# Autodesk Inventor assembly: Сборка
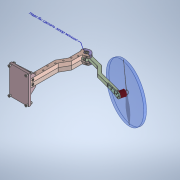
[picture p0: Inventor's stored thumbnail of the model, 180x180]
Saved by Autodesk Inventor 2021.2 (Build 252289000, 289)
## iProperties
Created: 2024-10-29
Part Number: Сборка
Document SubType Name: Assembly
Designer: barko
Author: barko
## Documents named in this file (24)
- C:\Users\DELL\Desktop\Personal\PID_controller\PID_controller\Mechanics\3D_model\Сборка.iam
- C:\Users\DELL\Desktop\Personal\PID_controller\PID_controller\Mechanics\3D_model\Ножка 1.ipt
- C:\Users\DELL\Desktop\Personal\PID_controller\PID_controller\Mechanics\3D_model\Ножка 2.ipt
- C:\Users\DELL\Desktop\Personal\PID_controller\PID_controller\Mechanics\3D_model\Скобка 1.ipt
- C:\Users\DELL\Desktop\Personal\PID_controller\PID_controller\Mechanics\3D_model\Скобка 2.ipt
- C:\Users\DELL\Desktop\Personal\PID_controller\PID_controller\Mechanics\3D_model\Фланец.ipt
- C:\Users\DELL\Desktop\Personal\PID_controller\PID_controller\Mechanics\3D_model\Луч.ipt
- C:\Users\DELL\Desktop\Personal\PID_controller\PID_controller\Mechanics\3D_model\Ложечка.ipt
- C:\Users\DELL\Desktop\Personal\PID_controller\PID_controller\Mechanics\3D_model\Моторчик.ipt
- C:\Users\DELL\Desktop\Personal\PID_controller\PID_controller\Mechanics\3D_model\Пропеллер.ipt
- C:\Users\DELL\Documents\Inventor\Content Center Files\R2021\ru-RU\GOST 11738-84\Винт M3-6gx30 ГОСТ 11738-84.ipt
- C:\Users\DELL\Documents\Inventor\Content Center Files\R2021\ru-RU\GOST 5916-70\Гайка M3-6H ГОСТ 5916-70.ipt
- C:\Users\DELL\Documents\Inventor\Content Center Files\R2021\ru-RU\Nut GOST 15524-70\Гайка M4-6H ГОСТ 15524-70.ipt
- C:\Users\DELL\Documents\Inventor\Content Center Files\R2021\ru-RU\GOST 11738-84\Винт M4-6gx25 ГОСТ 11738-84.ipt
- C:\Users\DELL\Documents\Inventor\Content Center Files\R2021\ru-RU\GOST 11738-84\Винт M4-6gx20 ГОСТ 11738-84.ipt
- C:\Users\DELL\Desktop\Personal\PID_controller\PID_controller\Mechanics\3D_model\Подшипник.ipt
- C:\Users\DELL\Documents\Inventor\Content Center Files\R2021\ru-RU\GOST 5915-70\Гайка M6-6H ГОСТ 5915-70(1).ipt
- C:\Users\DELL\Documents\Inventor\Content Center Files\R2021\ru-RU\GOST 11738-84\Винт M6-6gx50 ГОСТ 11738-84.ipt
- C:\Users\DELL\Documents\Inventor\Content Center Files\R2021\ru-RU\GOST 11738-84\Винт M6-6gx25 ГОСТ 11738-84.ipt
- C:\Users\DELL\Documents\Inventor\Content Center Files\R2021\ru-RU\GOST 11371-78  A\Шайба 6 ГОСТ 11371-78.ipt
- C:\Users\DELL\Documents\Inventor\Content Center Files\R2021\ru-RU\Washer 1 GOST 6402-78\Шайба 6Л ГОСТ 6402-78.ipt
- C:\Users\DELL\Documents\Inventor\Content Center Files\R2021\ru-RU\GOST 17475-80 (2)\Винт 2.M6-6gx30 ГОСТ 17475-80.ipt
- C:\Users\DELL\Documents\Inventor\Content Center Files\R2021\ru-RU\ISO 10642(1)\ISO 10642 - M3x8.ipt
- C:\Users\DELL\Documents\Inventor\Content Center Files\R2021\ru-RU\ISO 10642(1)\ISO 10642 - M3x12.ipt
## Components (68 placed, 23 different names)
1. Ножка 1:1 — Совмещение:1, Угол:1, Совмещение:2, Совмещение:3, Совмещение:4, Совмещение:5, Совмещение:6, Совмещение:7, Совмещение:8, Совмещение:9, Совмещение:10, Совмещение:11, Совмещение:12, Совмещение:13, Совмещение:14, Совмещение:15, Совмещение:16, Совмещение:18, Совмещение:20, Совмещение:22, Совмещение:24, Совмещение:26, Совмещение:28, Вставка:4, Совмещение:46, Совмещение:58, Совмещение:62, Совмещение:64
2. Ножка 2:1 — Совмещение:17, Совмещение:19, Совмещение:21, Совмещение:23, Совмещение:25, Совмещение:27, Совмещение:29, Вставка:5, Совмещение:59, Совмещение:60, Совмещение:63, Совмещение:65
3. Скобка 1:1 — Совмещение:42, Совмещение:43, Совмещение:44, Совмещение:53, Совмещение:54, Совмещение:55
4. Скобка 2:1 — Совмещение:47, Совмещение:48, Совмещение:49, Совмещение:50, Совмещение:51, Совмещение:52
5. Фланец:1 — Совмещение:66, Совмещение:67, Совмещение:68, Совмещение:69, Совмещение:70, Совмещение:71, Совмещение:72, Совмещение:73, Совмещение:74, Совмещение:75, Совмещение:76, Совмещение:77, Вставка:6, Вставка:7, Вставка:8, Вставка:9, Заподлицо:2, Заподлицо:3, Заподлицо:4, Заподлицо:5
6. Луч:1 — Заподлицо:1, Совмещение:1, Угол:1, Совмещение:37, Совмещение:38, Совмещение:40, Совмещение:41, Совмещение:95, Совмещение:96, Угол:2
7. Ложечка:1 — Вставка:1, Совмещение:86, Совмещение:87, Совмещение:88, Совмещение:89, Совмещение:90, Совмещение:91, Совмещение:92, Совмещение:93, Совмещение:94, Совмещение:96, Угол:2
8. Моторчик:1 — Вставка:1, Вставка:2, Совмещение:95
9. Пропеллер:1 — Вставка:2
10. Подшипник:1 — Вставка:4
11. Подшипник:2 — Вставка:5
12. Винт ГОСТ 11738-84 M 3x30:1 — Совмещение:2, Совмещение:3
13. Гайка ГОСТ 5916-70 M3:1 — Совмещение:16, Совмещение:17
14. Винт ГОСТ 11738-84 M 3x30:2 — Совмещение:4, Совмещение:5
15. Винт ГОСТ 11738-84 M 3x30:3 — Совмещение:6, Совмещение:7
16. Винт ГОСТ 11738-84 M 3x30:4 — Совмещение:8, Совмещение:9
17. Винт ГОСТ 11738-84 M 3x30:5 — Совмещение:10, Совмещение:11
18. Винт ГОСТ 11738-84 M 3x30:6 — Совмещение:12, Совмещение:13
19. Винт ГОСТ 11738-84 M 3x30:7 — Совмещение:14, Совмещение:15
20. Гайка ГОСТ 5916-70 M3:2 — Совмещение:18, Совмещение:19
21. Гайка ГОСТ 5916-70 M3:3 — Совмещение:20, Совмещение:21
22. Гайка ГОСТ 5916-70 M3:4 — Совмещение:22, Совмещение:23
23. Гайка ГОСТ 5916-70 M3:5 — Совмещение:24, Совмещение:25
24. Гайка ГОСТ 5916-70 M3:6 — Совмещение:26, Совмещение:27
25. Гайка ГОСТ 5916-70 M3:7 — Совмещение:28, Совмещение:29
26. Винт ГОСТ 11738-84 M 4x20:1 — Совмещение:45, Совмещение:46
27. Гайка ГОСТ 15524-70 M4:1 — Совмещение:42, Совмещение:43, Совмещение:44, Совмещение:45
28. Винт ГОСТ 11738-84 M 4x25:1 — Совмещение:37, Совмещение:39
29. Гайка ГОСТ 15524-70 M4:2 — Совмещение:38, Совмещение:39, Совмещение:40, Совмещение:41
30. Винт ГОСТ 11738-84 M 4x20:2 — Совмещение:56, Совмещение:58
31. Винт ГОСТ 11738-84 M 4x20:3 — Совмещение:60, Совмещение:61
32. Винт ГОСТ 11738-84 M 4x20:4 — Совмещение:57, Совмещение:59
33. Гайка ГОСТ 15524-70 M4:3 — Совмещение:47, Совмещение:48, Совмещение:49, Совмещение:61
34. Гайка ГОСТ 15524-70 M4:4 — Совмещение:53, Совмещение:54, Совмещение:55, Совмещение:56
35. Гайка ГОСТ 15524-70 M4:5 — Совмещение:50, Совмещение:51, Совмещение:52, Совмещение:57
36. Гайка ГОСТ 5915-70 M6:1 — Совмещение:69, Совмещение:72, Совмещение:73, Совмещение:80
37. Гайка ГОСТ 5915-70 M6:2 — Совмещение:71, Совмещение:74, Совмещение:75, Совмещение:81
38. Гайка ГОСТ 5915-70 M6:3 — Совмещение:70, Совмещение:76, Совмещение:77, Совмещение:79
39. Гайка ГОСТ 5915-70 M6:4 — Совмещение:66, Совмещение:67, Совмещение:68, Совмещение:78
40. Винт ГОСТ 11738-84 M 6x50:1 — Совмещение:64, Совмещение:79
41. Винт ГОСТ 11738-84 M 6x25:2 — Совмещение:63, Совмещение:80
42. Винт ГОСТ 11738-84 M 6x25:1 — Совмещение:62, Совмещение:78
43. Винт ГОСТ 11738-84 M 6x50:2 — Совмещение:65, Совмещение:81
44. Шайба  ГОСТ 11371-78 6,4:1 — Вставка:6, Вставка:10
45. Шайба  ГОСТ 11371-78 6,4:2 — Вставка:7, Вставка:11
46. Шайба  ГОСТ 11371-78 6,4:3 — Вставка:8, Вставка:13
47. Шайба  ГОСТ 11371-78 6,4:4 — Вставка:9, Вставка:12
48. Шайба 1 ГОСТ 6402-78 6Л:1 — Вставка:10, Вставка:16
49. Шайба 1 ГОСТ 6402-78 6Л:2 — Вставка:11, Вставка:15
50. Шайба 1 ГОСТ 6402-78 6Л:3 — Вставка:12, Вставка:17
51. Шайба 1 ГОСТ 6402-78 6Л:4 — Вставка:13, Вставка:14
52. Гайка ГОСТ 5915-70 M6:5 — Вставка:14, Совмещение:85
53. Гайка ГОСТ 5915-70 M6:6 — Вставка:15, Совмещение:84
54. Гайка ГОСТ 5915-70 M6:7 — Вставка:16, Совмещение:82
55. Гайка ГОСТ 5915-70 M6:8 — Вставка:17, Совмещение:83
56. Винт 2 ГОСТ 17475-80 M6 x 30:1 — Совмещение:82, Заподлицо:3
57. Винт 2 ГОСТ 17475-80 M6 x 30:2 — Совмещение:83, Заподлицо:2
58. Винт 2 ГОСТ 17475-80 M6 x 30:3 — Совмещение:85, Заподлицо:5
59. Винт 2 ГОСТ 17475-80 M6 x 30:4 — Совмещение:84, Заподлицо:4
60. ISO 10642 M3x12:1 — Совмещение:86
61. ISO 10642 M3x12:2 — Совмещение:87
62. ISO 10642 M3x12:3 — Совмещение:88
63. ISO 10642 M3x12:4 — Совмещение:89
64. ISO 10642 M3x12:5 — Совмещение:90
65. ISO 10642 M3x8:1 — Совмещение:91
66. ISO 10642 M3x8:2 — Совмещение:92
67. ISO 10642 M3x8:3 — Совмещение:93
68. ISO 10642 M3x8:4 — Совмещение:94
## Relationships (112: Mate 89, Insert 16, Flush 5, Angle 2)
- Вставка:1 [Insert]: Ложечка:1 ↔ Моторчик:1
- Вставка:2 [Insert] (2 mm): Моторчик:1 ↔ Пропеллер:1
- Заподлицо:1 [Flush]: Луч:1
- Совмещение:1 [Mate]: Ножка 1:1 ↔ Луч:1
- Угол:1 [Angle] (0 deg): Ножка 1:1 ↔ Луч:1
- Совмещение:2 [Mate]: Ножка 1:1 ↔ Винт ГОСТ 11738-84 M 3x30:1
- Совмещение:3 [Mate]: Ножка 1:1 ↔ Винт ГОСТ 11738-84 M 3x30:1
- Совмещение:4 [Mate]: Ножка 1:1 ↔ Винт ГОСТ 11738-84 M 3x30:2
- Совмещение:5 [Mate]: Ножка 1:1 ↔ Винт ГОСТ 11738-84 M 3x30:2
- Совмещение:6 [Mate]: Ножка 1:1 ↔ Винт ГОСТ 11738-84 M 3x30:3
- Совмещение:7 [Mate]: Ножка 1:1 ↔ Винт ГОСТ 11738-84 M 3x30:3
- Совмещение:8 [Mate]: Ножка 1:1 ↔ Винт ГОСТ 11738-84 M 3x30:4
- Совмещение:9 [Mate]: Ножка 1:1 ↔ Винт ГОСТ 11738-84 M 3x30:4
- Совмещение:10 [Mate]: Ножка 1:1 ↔ Винт ГОСТ 11738-84 M 3x30:5
- Совмещение:11 [Mate]: Ножка 1:1 ↔ Винт ГОСТ 11738-84 M 3x30:5
- Совмещение:12 [Mate]: Ножка 1:1 ↔ Винт ГОСТ 11738-84 M 3x30:6
- Совмещение:13 [Mate]: Ножка 1:1 ↔ Винт ГОСТ 11738-84 M 3x30:6
- Совмещение:14 [Mate]: Ножка 1:1 ↔ Винт ГОСТ 11738-84 M 3x30:7
- Совмещение:15 [Mate]: Ножка 1:1 ↔ Винт ГОСТ 11738-84 M 3x30:7
- Совмещение:16 [Mate]: Ножка 1:1 ↔ Гайка ГОСТ 5916-70 M3:1
- Совмещение:17 [Mate]: Ножка 2:1 ↔ Гайка ГОСТ 5916-70 M3:1
- Совмещение:18 [Mate]: Ножка 1:1 ↔ Гайка ГОСТ 5916-70 M3:2
- Совмещение:19 [Mate]: Ножка 2:1 ↔ Гайка ГОСТ 5916-70 M3:2
- Совмещение:20 [Mate]: Ножка 1:1 ↔ Гайка ГОСТ 5916-70 M3:3
- Совмещение:21 [Mate]: Ножка 2:1 ↔ Гайка ГОСТ 5916-70 M3:3
- Совмещение:22 [Mate]: Ножка 1:1 ↔ Гайка ГОСТ 5916-70 M3:4
- Совмещение:23 [Mate]: Ножка 2:1 ↔ Гайка ГОСТ 5916-70 M3:4
- Совмещение:24 [Mate]: Ножка 1:1 ↔ Гайка ГОСТ 5916-70 M3:5
- Совмещение:25 [Mate]: Ножка 2:1 ↔ Гайка ГОСТ 5916-70 M3:5
- Совмещение:26 [Mate]: Ножка 1:1 ↔ Гайка ГОСТ 5916-70 M3:6
- Совмещение:27 [Mate]: Ножка 2:1 ↔ Гайка ГОСТ 5916-70 M3:6
- Совмещение:28 [Mate]: Ножка 1:1 ↔ Гайка ГОСТ 5916-70 M3:7
- Совмещение:29 [Mate]: Ножка 2:1 ↔ Гайка ГОСТ 5916-70 M3:7
- Совмещение:37 [Mate]: Луч:1 ↔ Винт ГОСТ 11738-84 M 4x25:1
- Совмещение:38 [Mate]: Луч:1 ↔ Гайка ГОСТ 15524-70 M4:2
- Совмещение:39 [Mate]: Винт ГОСТ 11738-84 M 4x25:1 ↔ Гайка ГОСТ 15524-70 M4:2
- Совмещение:40 [Mate]: Луч:1 ↔ Гайка ГОСТ 15524-70 M4:2
- Совмещение:41 [Mate]: Луч:1 ↔ Гайка ГОСТ 15524-70 M4:2
- Вставка:4 [Insert]: Ножка 1:1 ↔ Подшипник:1
- Вставка:5 [Insert]: Ножка 2:1 ↔ Подшипник:2
- Совмещение:42 [Mate]: Скобка 1:1 ↔ Гайка ГОСТ 15524-70 M4:1
- Совмещение:43 [Mate]: Скобка 1:1 ↔ Гайка ГОСТ 15524-70 M4:1
- Совмещение:44 [Mate]: Скобка 1:1 ↔ Гайка ГОСТ 15524-70 M4:1
- Совмещение:45 [Mate]: Винт ГОСТ 11738-84 M 4x20:1 ↔ Гайка ГОСТ 15524-70 M4:1
- Совмещение:46 [Mate]: Ножка 1:1 ↔ Винт ГОСТ 11738-84 M 4x20:1
- Совмещение:47 [Mate]: Скобка 2:1 ↔ Гайка ГОСТ 15524-70 M4:3
- Совмещение:48 [Mate]: Скобка 2:1 ↔ Гайка ГОСТ 15524-70 M4:3
- Совмещение:49 [Mate]: Скобка 2:1 ↔ Гайка ГОСТ 15524-70 M4:3
- Совмещение:50 [Mate]: Скобка 2:1 ↔ Гайка ГОСТ 15524-70 M4:5
- Совмещение:51 [Mate]: Скобка 2:1 ↔ Гайка ГОСТ 15524-70 M4:5
- Совмещение:52 [Mate]: Скобка 2:1 ↔ Гайка ГОСТ 15524-70 M4:5
- Совмещение:53 [Mate]: Скобка 1:1 ↔ Гайка ГОСТ 15524-70 M4:4
- Совмещение:54 [Mate]: Скобка 1:1 ↔ Гайка ГОСТ 15524-70 M4:4
- Совмещение:55 [Mate]: Скобка 1:1 ↔ Гайка ГОСТ 15524-70 M4:4
- Совмещение:56 [Mate]: Винт ГОСТ 11738-84 M 4x20:2 ↔ Гайка ГОСТ 15524-70 M4:4
- Совмещение:57 [Mate]: Винт ГОСТ 11738-84 M 4x20:4 ↔ Гайка ГОСТ 15524-70 M4:5
- Совмещение:58 [Mate]: Ножка 1:1 ↔ Винт ГОСТ 11738-84 M 4x20:2
- Совмещение:59 [Mate]: Ножка 2:1 ↔ Винт ГОСТ 11738-84 M 4x20:4
- Совмещение:60 [Mate]: Ножка 2:1 ↔ Винт ГОСТ 11738-84 M 4x20:3
- Совмещение:61 [Mate]: Винт ГОСТ 11738-84 M 4x20:3 ↔ Гайка ГОСТ 15524-70 M4:3
- Совмещение:62 [Mate]: Ножка 1:1 ↔ Винт ГОСТ 11738-84 M 6x25:1
- Совмещение:63 [Mate]: Ножка 2:1 ↔ Винт ГОСТ 11738-84 M 6x25:2
- Совмещение:64 [Mate]: Ножка 1:1 ↔ Винт ГОСТ 11738-84 M 6x50:1
- Совмещение:65 [Mate]: Ножка 2:1 ↔ Винт ГОСТ 11738-84 M 6x50:2
- Совмещение:66 [Mate]: Фланец:1 ↔ Гайка ГОСТ 5915-70 M6:4
- Совмещение:67 [Mate]: Фланец:1 ↔ Гайка ГОСТ 5915-70 M6:4
- Совмещение:68 [Mate]: Фланец:1 ↔ Гайка ГОСТ 5915-70 M6:4
- Совмещение:69 [Mate]: Фланец:1 ↔ Гайка ГОСТ 5915-70 M6:1
- Совмещение:70 [Mate]: Фланец:1 ↔ Гайка ГОСТ 5915-70 M6:3
- Совмещение:71 [Mate]: Фланец:1 ↔ Гайка ГОСТ 5915-70 M6:2
- Совмещение:72 [Mate]: Фланец:1 ↔ Гайка ГОСТ 5915-70 M6:1
- Совмещение:73 [Mate]: Фланец:1 ↔ Гайка ГОСТ 5915-70 M6:1
- Совмещение:74 [Mate]: Фланец:1 ↔ Гайка ГОСТ 5915-70 M6:2
- Совмещение:75 [Mate]: Фланец:1 ↔ Гайка ГОСТ 5915-70 M6:2
- Совмещение:76 [Mate]: Фланец:1 ↔ Гайка ГОСТ 5915-70 M6:3
- Совмещение:77 [Mate]: Фланец:1 ↔ Гайка ГОСТ 5915-70 M6:3
- Совмещение:78 [Mate]: Гайка ГОСТ 5915-70 M6:4 ↔ Винт ГОСТ 11738-84 M 6x25:1
- Совмещение:79 [Mate]: Гайка ГОСТ 5915-70 M6:3 ↔ Винт ГОСТ 11738-84 M 6x50:1
- Совмещение:80 [Mate]: Гайка ГОСТ 5915-70 M6:1 ↔ Винт ГОСТ 11738-84 M 6x25:2
- Совмещение:81 [Mate]: Гайка ГОСТ 5915-70 M6:2 ↔ Винт ГОСТ 11738-84 M 6x50:2
- Вставка:6 [Insert]: Фланец:1 ↔ Шайба  ГОСТ 11371-78 6,4:1
- Вставка:7 [Insert]: Фланец:1 ↔ Шайба  ГОСТ 11371-78 6,4:2
- Вставка:8 [Insert]: Фланец:1 ↔ Шайба  ГОСТ 11371-78 6,4:3
- Вставка:9 [Insert]: Фланец:1 ↔ Шайба  ГОСТ 11371-78 6,4:4
- Вставка:10 [Insert]: Шайба  ГОСТ 11371-78 6,4:1 ↔ Шайба 1 ГОСТ 6402-78 6Л:1
- Вставка:11 [Insert]: Шайба  ГОСТ 11371-78 6,4:2 ↔ Шайба 1 ГОСТ 6402-78 6Л:2
- Вставка:12 [Insert]: Шайба  ГОСТ 11371-78 6,4:4 ↔ Шайба 1 ГОСТ 6402-78 6Л:3
- Вставка:13 [Insert]: Шайба  ГОСТ 11371-78 6,4:3 ↔ Шайба 1 ГОСТ 6402-78 6Л:4
- Вставка:14 [Insert]: Шайба 1 ГОСТ 6402-78 6Л:4 ↔ Гайка ГОСТ 5915-70 M6:5
- Вставка:15 [Insert]: Шайба 1 ГОСТ 6402-78 6Л:2 ↔ Гайка ГОСТ 5915-70 M6:6
- Вставка:16 [Insert]: Шайба 1 ГОСТ 6402-78 6Л:1 ↔ Гайка ГОСТ 5915-70 M6:7
- Вставка:17 [Insert]: Шайба 1 ГОСТ 6402-78 6Л:3 ↔ Гайка ГОСТ 5915-70 M6:8
- Совмещение:82 [Mate]: Гайка ГОСТ 5915-70 M6:7 ↔ Винт 2 ГОСТ 17475-80 M6 x 30:1
- Совмещение:83 [Mate]: Гайка ГОСТ 5915-70 M6:8 ↔ Винт 2 ГОСТ 17475-80 M6 x 30:2
- Совмещение:84 [Mate]: Гайка ГОСТ 5915-70 M6:6 ↔ Винт 2 ГОСТ 17475-80 M6 x 30:4
- Совмещение:85 [Mate]: Гайка ГОСТ 5915-70 M6:5 ↔ Винт 2 ГОСТ 17475-80 M6 x 30:3
- Заподлицо:2 [Flush] (9 mm): Фланец:1 ↔ Винт 2 ГОСТ 17475-80 M6 x 30:2
- Заподлицо:3 [Flush] (9 mm): Фланец:1 ↔ Винт 2 ГОСТ 17475-80 M6 x 30:1
- Заподлицо:4 [Flush] (9 mm): Фланец:1 ↔ Винт 2 ГОСТ 17475-80 M6 x 30:4
- Заподлицо:5 [Flush] (9 mm): Фланец:1 ↔ Винт 2 ГОСТ 17475-80 M6 x 30:3
- Совмещение:86 [Mate]: Ложечка:1 ↔ ISO 10642 M3x12:1
- Совмещение:87 [Mate]: Ложечка:1 ↔ ISO 10642 M3x12:2
- Совмещение:88 [Mate]: Ложечка:1 ↔ ISO 10642 M3x12:3
- Совмещение:89 [Mate]: Ложечка:1 ↔ ISO 10642 M3x12:4
- Совмещение:90 [Mate]: Ложечка:1 ↔ ISO 10642 M3x12:5
- Совмещение:91 [Mate]: Ложечка:1 ↔ ISO 10642 M3x8:1
- Совмещение:92 [Mate]: Ложечка:1 ↔ ISO 10642 M3x8:2
- Совмещение:93 [Mate]: Ложечка:1 ↔ ISO 10642 M3x8:3
- Совмещение:94 [Mate]: Ложечка:1 ↔ ISO 10642 M3x8:4
- Совмещение:95 [Mate]: Луч:1 ↔ Моторчик:1
- Совмещение:96 [Mate]: Луч:1 ↔ Ложечка:1
- Угол:2 [Angle] (180 deg): Луч:1 ↔ Ложечка:1
